# Autodesk Inventor assembly: hegnspæl omvendt
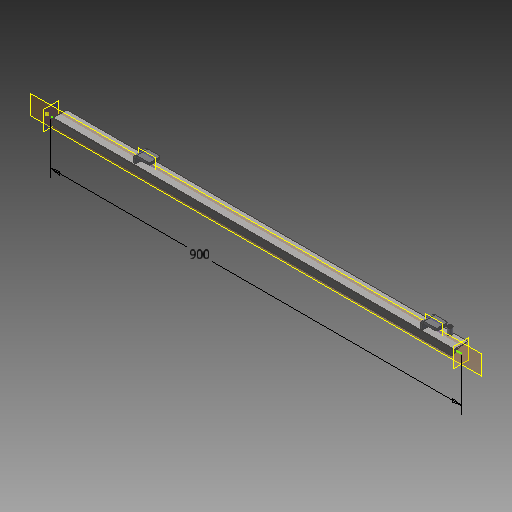
[picture p0: Inventor's stored thumbnail of the model, 512x512]
Saved by Autodesk Inventor 2018 (Build 220112000, 112)
## iProperties
Created: 2019-09-30
Part Number: hegnspæl omvendt
Document SubType Name: Assembly
Designer: gust3763
Mass: 1821.47 g
Surface Area: 1100.09 cm^2
Volume: 232.034 cm^3
Density: 7.85 g/cm^3
_SolveAssemblyDoc: Frame Generator Solve Assembly
_Version: 15.0.0
Author: gust3763
## Documents named in this file (8)
- Z:\trappe\hegn\hegnspæl omvendt.iam
- hegnspæl omvendt.iam
- Z:\trappe\hegn\t-profil.ipt
- Z:\trappe\hegn\t-profil\Frame\Frame0002.iam
- Z:\trappe\hegn\hage.ipt
- Z:\trappe\hegn\gevindmuffe.ipt
- C:\Users\loppen\Documents\Inventor\Content Center Files\R2018\en-US\ISO 4762(2)\ISO 4762 - M6 x 16ISO.ipt
- Z:\trappe\trappe.xlsx
## Components (6 placed, 5 different names)
1. t-profil:1
2. Frame0002:1 [sub-assembly] — Mate:1, Mate:2, Mate:3, Angle:1, Mate:4, Angle:2, Mate:5, Angle:3, Flush:5, Flush:6, Mate:6, Mate:7, Mate:8, Mate:10
3. hage:1 — Mate:1, Flush:5, Flush:7, Mate:6
4. hage:2 — Mate:2, Flush:6, Flush:7
5. gevindmuffe:1 — Mate:7, Mate:8, Mate:9
6. ISO 4762 M6 x 16:1 — Mate:9, Mate:10
## Relationships (16: Mate 10, Angle 3, Flush 3)
- Mate:1: Frame0002:1 ↔ hage:1
- Mate:2: Frame0002:1 ↔ hage:2
- Mate:3: Frame0002:1
- Angle:1 (0 deg): Frame0002:1
- Mate:4: Frame0002:1
- Angle:2 (0 deg): Frame0002:1
- Mate:5: Frame0002:1
- Angle:3 (0 deg): Frame0002:1
- Flush:5 (2.5 mm): Frame0002:1 ↔ hage:1
- Flush:6 (2.5 mm): Frame0002:1 ↔ hage:2
- Flush:7 (630 mm): hage:1 ↔ hage:2
- Mate:6 (-178 mm): Frame0002:1 ↔ hage:1
- Mate:7: Frame0002:1 ↔ gevindmuffe:1
- Mate:8: Frame0002:1 ↔ gevindmuffe:1
- Mate:9: gevindmuffe:1 ↔ ISO 4762 M6 x 16:1
- Mate:10: Frame0002:1 ↔ ISO 4762 M6 x 16:1
## Named parameters: trappevinkel = 34.3 deg, trappestifter_dia = 25 mm, trappestifter_huldia = 25.8 mm, trappestifter_skraa_huldia = 26.6 mm, trappestifter_laengde = 228 mm, perforeringsbredde = 6 mm, perforeringshulprocent = 80 mm, perforeringshullaengde = 62.8 mm, perforeringshullaengde_top = 61 mm, perforeringshullaengde_bund = 61.6 mm, perforeringsoffset = 8 mm, perforeringsoffset_top = 8 mm, perforeringsoffset_bund = 8 mm, laskehul_dia = 13 mm, haandfang_offset_fra_top = 90 mm, balusterhul_udvidelse = 1 mm, pladetykkelse = 3 mm, trinhoejde = 100 mm, trinbredde = 1884 mm
